# Autodesk Inventor assembly: 모서리 결합 조립
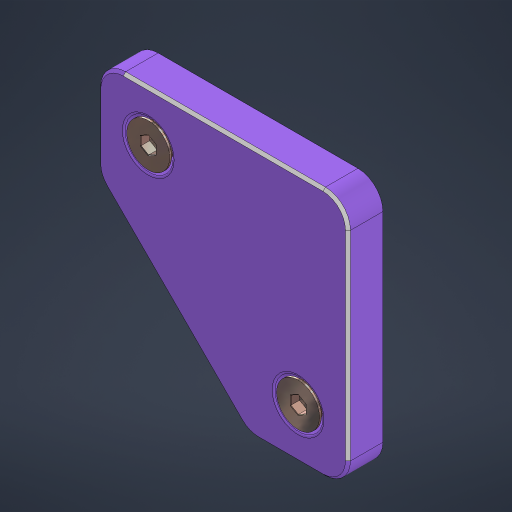
[picture p0: Inventor's stored thumbnail of the model, 512x512]
Saved by Autodesk Inventor 2024 (Build 280153000, 153)
## iProperties
Created: 2024-01-12
Part Number: 모서리 결합 조립
Document SubType Name: Assembly
Designer: KBU
Author: KBU
## Documents named in this file (3)
- D:\모델링\챔버\모서리 결합 조립.iam
- D:\모델링\챔버\모서리 결합 수정.ipt
- D:\모델링\챔버\M5 접시머리 나사.ipt
## Components (3 placed, 2 different names)
1. 모서리 결합 수정:1 — 삽입:1, 삽입:2
2. M5 접시머리 나사:1 — 삽입:1
3. M5 접시머리 나사:2 — 삽입:2
## Relationships (2: Insert 2)
- 삽입:1 [Insert]: 모서리 결합 수정:1 ↔ M5 접시머리 나사:1
- 삽입:2 [Insert]: 모서리 결합 수정:1 ↔ M5 접시머리 나사:2
